# Autodesk Inventor assembly: FullAssem
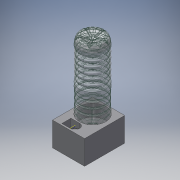
[picture p0: Inventor's stored thumbnail of the model, 180x180]
Saved by Autodesk Inventor 2019 (Build 230136000, 136)
## iProperties
Created: 2019-04-09
Part Number: FullAssem
Document SubType Name: Assembly
Designer: Jorian Brusind
Author: Jorian Brusind
## Documents named in this file (4)
- C:\Users\Jorian Brusind\Documents\GitHub\PersonalProjects\Automated Terrarium Project\Inventor Files\V3\FullAssem.iam
- C:\Users\Jorian Brusind\Documents\GitHub\PersonalProjects\Automated Terrarium Project\Inventor Files\V3\mini_pump.ipt
- C:\Users\Jorian Brusind\Documents\GitHub\PersonalProjects\Automated Terrarium Project\Inventor Files\V3\Bottle 600ml.iam
- C:\Users\Jorian Brusind\Documents\GitHub\PersonalProjects\Automated Terrarium Project\Inventor Files\V3\BoitCase.ipt
## Components (3 placed, 3 different names)
1. Bottle 600ml:1 [sub-assembly] — Mate:1
2. BoitCase:1 — Mate:1, Mate:2, Mate:3
3. mini_pump:1 — Mate:2, Mate:3
## Relationships (3: Mate 3)
- Mate:1: Bottle 600ml:1 ↔ BoitCase:1
- Mate:2: BoitCase:1 ↔ mini_pump:1
- Mate:3: BoitCase:1 ↔ mini_pump:1
